# Autodesk Inventor assembly: 1301.000(1)
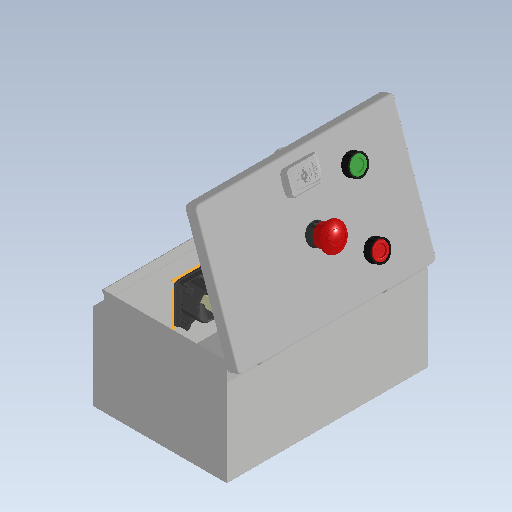
[picture p0: Inventor's stored thumbnail of the model, 512x512]
Saved by Autodesk Inventor 2025.2 (Build 292293000, 293)
## iProperties
Category: PARTsolutions
Company: RITTAL
Created: 2025-05-02
Part Number: 1301.000(1)
Catalog Web Link: www.cadenas.de
Description: KX E-Box-stainless steel
Vendor: RITTAL
Document SubType Name: Assembly
Designer: psAdmin
Manufacturer: RITTAL
Mass: 539.801 g
Surface Area: 7071.18 cm^2
Volume: 539.801 cm^3
PSOL_IDENT_0: {$CADENAS_DATA/23d-libs/rittal/schaltschranksys/edelstahl/kleingehause/eb_edel_2_0_asmtab.prj},188 {
PSOL_IDENT_1: VTYP=3D},{STYP=ASSTAB},{NB=1301.000(1)},{LINA=1301.000},{NN=KX E-Box},{DATE=28.04.2025 21:10:46},{GE
PSOL_IDENT_2: OMDATE=11.04.2025 11:21:28},{VERSION=},{LINEID=690},{WBVAR=DETAIL},{WBNUMERIC=DETAIL}  {NB=1301.000(
PSOL_IDENT_3: 1)},{LINA=1301.000},{KT=DUMMY},{BEST=1301.000},{INFOPAGE=-},{DETAIL=1},{INFOWWW=Website},{BEZ1=KX El
PSOL_IDENT_4: ektronik-Box},{BEZ2=Edelstahl, 1.4404},{BEZ3=eintürig},{B=200},{H=300},{T=155},{F=175},{G=285},{GEW=
PSOL_IDENT_5: 3,889},{INFOPATH=http://www.rittal.com/com-en/part/1301000},{CNSECLASS51=27-18-01-02},{CNSECLASS70=2
PSOL_IDENT_6: 7-18-01-01},{CNSECLASS80=27-18-01-01},{CNSETIM40=EC002713},{PPATH=assemblies_eb_edel_2_0/kx_eb_edel_
PSOL_IDENT_7: new_asmtpl.prj},{BESTE1=1301},{BESTE2=000},{CNSETIM80=EC000261},{CNSETIM90=EC000261},{CNSECLASS60=27
PSOL_IDENT_8: -18-01-01},{UNSPSC=31-26-15-02}
NB: 1301.000(1)
NN: KX E-Box
NT: stainless steel
NBSYN: $BEST.($DETAIL.)
LINA: 1301.000
CATALOG: Rittal
BEST: 1301.000
DETAIL: high
INFOWWW: Website
BEZ1: KX E-Box
BEZ2: Stainless steel, 1.4404
BEZ3: single door
B: 200
H: 300
T: 155
F: 175
G: 285
CNSECLASS70: 27-18-01-01
CNSECLASS80: 27-18-01-01
CNSETIM80: EC000261
CNSETIM90: EC000261
CNSECLASS60: 27-18-01-01
UNSPSC: 31-26-15-02
SUPPLIER: RITTAL
ARTICLENO: 1301.000(1)
BOMINFO: 1301.000
CREATOR: CADENAS GmbH
Title: 1301.000
Author: Cadenas PARTsolutions
Comments: stainless steel
## Documents named in this file (22)
- C:\Users\Gustavo Sousa\Downloads\Inventor\design\quadro_eletrico\AIS2024\1301_000_1_\1301_000(1).iam
- C:\Users\Gustavo Sousa\Downloads\Inventor\design\quadro_eletrico\AIS2024\1301_000_1_\1301_000_1_(1).ipt
- C:\Users\Gustavo Sousa\Downloads\Inventor\design\quadro_eletrico\AIS2024\1301_000_1_\1301_000_6_(1).ipt
- C:\Users\Gustavo Sousa\Downloads\Inventor\design\quadro_eletrico\AIS2024\1301_000_1_\1301_000_4_(1).ipt
- C:\Users\Gustavo Sousa\Downloads\Inventor\design\quadro_eletrico\AIS2024\1301_000_1_\1301_000_2_(1).ipt
- C:\Users\Gustavo Sousa\Downloads\Inventor\design\quadro_eletrico\AIS2024\1301_000_1_\1301_000_5_(1).ipt
- C:\Users\Gustavo Sousa\Downloads\Inventor\design\quadro_eletrico\AIS2024\1301_000_1_\1301_000_3_(1).ipt
- C:\Users\Gustavo Sousa\Downloads\Inventor\design\quadro_eletrico\AIS2024\1301_000_1_\1301_000_10_(1).ipt
- C:\Users\Gustavo Sousa\Downloads\Inventor\design\calhadine\PP0735H(1).ipt
- C:\Users\Gustavo Sousa\Downloads\Inventor\design\disjuntores\Diferencial\CFC 225P\CFC 225P v16\CFC 225P v16\CFC 225P v16.ipt
- C:\Users\Gustavo Sousa\Downloads\Inventor\design\disjuntores\Polares\SD C25 1P - STECK\SD C25 1P - STECK\SD C25 1P - STECK.ipt
- C:\Users\Gustavo Sousa\Downloads\Inventor\design\barramento\MONTAGEM BARRAMENTO 10 FUROS NEUTRO\MONTAGEM BARRAMENTO 10 FUROS NEUTRO\MONTAGEM BARRAMENTO 10 FUROS NEUTRO.ipt
- C:\Users\Gustavo Sousa\Downloads\Inventor\design\barramento\BARRAMENTO 10 FUROS NEUTRO\BARRAMENTO 10 FUROS NEUTRO\BARRAMENTO 10 FUROS NEUTRO.ipt
- C:\Users\Gustavo Sousa\Downloads\Inventor\design\disjuntores\Motor\3RV24111AA200DA0.ipt
- C:\Users\Gustavo Sousa\Downloads\Inventor\design\corte_Geral\AIS2024\5SP33253.iam
- C:\Users\Gustavo Sousa\Downloads\Inventor\design\bornes\280-607_HI_0001_002.ipt
- C:\Users\Gustavo Sousa\Downloads\Inventor\design\bornes\280-607_HI.ipt
- C:\Users\Gustavo Sousa\Downloads\Inventor\design\bornes\280-607_HI_0003_001.ipt
- C:\Users\Gustavo Sousa\Downloads\Inventor\design\botões\P20BKR1\P20BKR1\P20BKR1.ipt
- C:\Users\Gustavo Sousa\Downloads\Inventor\design\botões\botao-lk2-ea42-verde-1nf-cod-14010-1.snapshot.1\MONTAGEM DO BOTÃO3.iam
- C:\Users\Gustavo Sousa\Downloads\Inventor\design\botões\botao-lk2-ea42-vermelho-1.snapshot.1\MONTAGEM DO BOTÃO.iam
- C:\Users\Gustavo Sousa\Downloads\Inventor\design\corte_Geral\eaton-main-switch-p1-25-m4-svb-switch-1.snapshot.1\Eaton main switch P1-25-M4-SVB - switch\Eaton main switch P1-25-M4-SVB - switch\Eaton main switch .ipt
## Components (31 placed, 26 different names)
1. 1301_000_1_(1):1 — to_MP_XY@1 <-> MONTAGEPLATTE_XY@2, to_MP_Z@1 <-> MONTAGEPLATTE_Z@2, to_MP_YZ@1 <-> MONTAGEPLATTE_YZ@2, to_HINGE_1_XY@1 <-> HINGE_XY@3, to_HINGE_1_Z@1 <-> HINGE_Z@3, to_HINGE_1_YZ@1 <-> HINGE_YZ@3, to_HINGE_2_XY@1 <-> HINGE_XY@4, to_HINGE_2_Z@1 <-> HINGE_Z@4, to_HINGE_2_YZ@1 <-> HINGE_YZ@4, to_L_Winkel_Bottom_XY@1 <-> SEITENTEIL_XY@7, to_L_Winkel_Bottom_Z@1 <-> SEITENTEIL_Z@7, to_L_Winkel_Bottom_YZ@1 <-> SEITENTEIL_YZ@7, to_L_Winkel_Top_XY@1 <-> SEITENTEIL_XY@10, to_L_Winkel_Top_Z@1 <-> SEITENTEIL_Z@10, to_L_Winkel_Top_YZ@1 <-> SEITENTEIL_YZ@10, Coincidente:67, Coincidente:68, Coincidente:69
2. 1301_000_6_(1):1 — to_MP_XY@1 <-> MONTAGEPLATTE_XY@2, to_MP_Z@1 <-> MONTAGEPLATTE_Z@2, to_MP_YZ@1 <-> MONTAGEPLATTE_YZ@2, Coincidente:23, Coincidente:24, Coincidente:25, Coincidente:26, Coincidente:27, Coincidente:28
3. 1301_000_4_(1):1 — to_HINGE_1_XY@1 <-> HINGE_XY@3, to_HINGE_1_Z@1 <-> HINGE_Z@3, to_HINGE_1_YZ@1 <-> HINGE_YZ@3
4. 1301_000_4_(1):2 — to_HINGE_2_XY@1 <-> HINGE_XY@4, to_HINGE_2_Z@1 <-> HINGE_Z@4, to_HINGE_2_YZ@1 <-> HINGE_YZ@4, DECKEL_XY@4 <-> to_HINGE_1_XY@5, DECKEL_Z@4 <-> to_HINGE_1_Z@5
5. 1301_000_2_(1):1 — DECKEL_XY@4 <-> to_HINGE_1_XY@5, DECKEL_Z@4 <-> to_HINGE_1_Z@5, VB_XY@5 <-> VV_XY@6, VB_Z@5 <-> VV_Z@6, VB_YZ@5 <-> VV_YZ@6, Coincidente:61, Coincidente:62, Coincidente:63, Coincidente:64, Coincidente:65, Coincidente:66
6. 1301_000_5_(1):1 — VB_XY@5 <-> VV_XY@6, VB_Z@5 <-> VV_Z@6, VB_YZ@5 <-> VV_YZ@6
7. 1301_000_3_(1):1 — to_L_Winkel_Bottom_XY@1 <-> SEITENTEIL_XY@7, to_L_Winkel_Bottom_Z@1 <-> SEITENTEIL_Z@7, to_L_Winkel_Bottom_YZ@1 <-> SEITENTEIL_YZ@7, SC1_XY@7 <-> SCHRAUBE_XY@8, SC1_Z@7 <-> SCHRAUBE_Z@8, SC1_YZ@7 <-> SCHRAUBE_YZ@8, SC2_XY@7 <-> SCHRAUBE_XY@9, SC2_Z@7 <-> SCHRAUBE_Z@9, SC2_YZ@7 <-> SCHRAUBE_YZ@9
8. 1301_000_10_(1):1 — SC1_XY@7 <-> SCHRAUBE_XY@8, SC1_Z@7 <-> SCHRAUBE_Z@8, SC1_YZ@7 <-> SCHRAUBE_YZ@8
9. 1301_000_10_(1):2 — SC2_XY@7 <-> SCHRAUBE_XY@9, SC2_Z@7 <-> SCHRAUBE_Z@9, SC2_YZ@7 <-> SCHRAUBE_YZ@9
10. 1301_000_3_(1):2 — to_L_Winkel_Top_XY@1 <-> SEITENTEIL_XY@10, to_L_Winkel_Top_Z@1 <-> SEITENTEIL_Z@10, to_L_Winkel_Top_YZ@1 <-> SEITENTEIL_YZ@10, SC1_XY@10 <-> SCHRAUBE_XY@11, SC1_Z@10 <-> SCHRAUBE_Z@11, SC1_YZ@10 <-> SCHRAUBE_YZ@11, SC2_XY@10 <-> SCHRAUBE_XY@12, SC2_Z@10 <-> SCHRAUBE_Z@12, SC2_YZ@10 <-> SCHRAUBE_YZ@12
11. 1301_000_10_(1):3 — SC1_XY@10 <-> SCHRAUBE_XY@11, SC1_Z@10 <-> SCHRAUBE_Z@11, SC1_YZ@10 <-> SCHRAUBE_YZ@11
12. 1301_000_10_(1):4 — SC2_XY@10 <-> SCHRAUBE_XY@12, SC2_Z@10 <-> SCHRAUBE_Z@12, SC2_YZ@10 <-> SCHRAUBE_YZ@12
13. calhadine 1 — Coincidente:23, Coincidente:24, Coincidente:25, Coincidente:29, Coincidente:30, Coincidente:31, Coincidente:32, Coincidente:33, Coincidente:34, Coincidente:35, Coincidente:36, Coincidente:37, Coincidente:38, Coincidente:39, Coincidente:40, Coincidente:41, Coincidente:42
14. calhadine 2 — Coincidente:26, Coincidente:27, Coincidente:28, Coincidente:44, Coincidente:45, Coincidente:46, Coincidente:47, Coincidente:49, Coincidente:50, Coincidente:52, Coincidente:53, Coincidente:55, Coincidente:56, Coincidente:57, Coincidente:58, Coincidente:59
15. disjuntor_diferencial — Coincidente:29, Coincidente:30
16. disjuntor_monopolar — Coincidente:31, Coincidente:32
17. barramento_Fase — Coincidente:33, Coincidente:34
18. barramento_Neutro — Coincidente:35, Coincidente:36
19. disjuntor_Motor1 — Coincidente:37, Coincidente:38
20. corte_Geral [sub-assembly] — Coincidente:39, Coincidente:40
21. disjuntor_Motor2 — Coincidente:41, Coincidente:42
22. borne_Viking_Neutro_1.0 — Coincidente:46, Coincidente:47, Coincidente:54
23. borne_Viking_Neutro_2.0 — Coincidente:52, Coincidente:53, Coincidente:54
24. borne_Viking_Fase_2 — Coincidente:44, Coincidente:45, Coincidente:51
25. borne_Viking_Fase_2.1 — Coincidente:49, Coincidente:50, Coincidente:51
26. borne_Viking_Terra_1.0 — Coincidente:55, Coincidente:56, Coincidente:57, Coincidente:60
27. borne_Viking_terra_1.1 — Coincidente:58, Coincidente:59, Coincidente:60
28. botao_emergencia — Coincidente:61, Coincidente:62
29. MONTAGEM DO BOTÃO3:1 [sub-assembly] — Coincidente:63, Coincidente:64
30. MONTAGEM DO BOTÃO:1 [sub-assembly] — Coincidente:65, Coincidente:66
31. Eaton main switch :1 — Coincidente:67, Coincidente:68, Coincidente:69
## Relationships (77: Mate 67, Angle 10)
- to_MP_XY@1 <-> MONTAGEPLATTE_XY@2 [Mate]: 1301_000_1_(1):1 ↔ 1301_000_6_(1):1
- to_MP_Z@1 <-> MONTAGEPLATTE_Z@2 [Mate]: 1301_000_1_(1):1 ↔ 1301_000_6_(1):1
- to_MP_YZ@1 <-> MONTAGEPLATTE_YZ@2 [Angle] (0 deg): 1301_000_1_(1):1 ↔ 1301_000_6_(1):1
- to_HINGE_1_XY@1 <-> HINGE_XY@3 [Mate]: 1301_000_1_(1):1 ↔ 1301_000_4_(1):1
- to_HINGE_1_Z@1 <-> HINGE_Z@3 [Mate]: 1301_000_1_(1):1 ↔ 1301_000_4_(1):1
- to_HINGE_1_YZ@1 <-> HINGE_YZ@3 [Angle] (90 deg): 1301_000_1_(1):1 ↔ 1301_000_4_(1):1
- to_HINGE_2_XY@1 <-> HINGE_XY@4 [Mate]: 1301_000_1_(1):1 ↔ 1301_000_4_(1):2
- to_HINGE_2_Z@1 <-> HINGE_Z@4 [Mate]: 1301_000_1_(1):1 ↔ 1301_000_4_(1):2
- to_HINGE_2_YZ@1 <-> HINGE_YZ@4 [Angle] (90 deg): 1301_000_1_(1):1 ↔ 1301_000_4_(1):2
- DECKEL_XY@4 <-> to_HINGE_1_XY@5 [Mate]: 1301_000_4_(1):2 ↔ 1301_000_2_(1):1
- DECKEL_Z@4 <-> to_HINGE_1_Z@5 [Mate]: 1301_000_4_(1):2 ↔ 1301_000_2_(1):1
- VB_XY@5 <-> VV_XY@6 [Mate]: 1301_000_2_(1):1 ↔ 1301_000_5_(1):1
- VB_Z@5 <-> VV_Z@6 [Mate]: 1301_000_2_(1):1 ↔ 1301_000_5_(1):1
- VB_YZ@5 <-> VV_YZ@6 [Angle] (0 deg): 1301_000_2_(1):1 ↔ 1301_000_5_(1):1
- to_L_Winkel_Bottom_XY@1 <-> SEITENTEIL_XY@7 [Mate] (-0.25 mm): 1301_000_1_(1):1 ↔ 1301_000_3_(1):1
- to_L_Winkel_Bottom_Z@1 <-> SEITENTEIL_Z@7 [Mate]: 1301_000_1_(1):1 ↔ 1301_000_3_(1):1
- to_L_Winkel_Bottom_YZ@1 <-> SEITENTEIL_YZ@7 [Angle] (-90 deg): 1301_000_1_(1):1 ↔ 1301_000_3_(1):1
- SC1_XY@7 <-> SCHRAUBE_XY@8 [Mate] (-1.575 mm): 1301_000_3_(1):1 ↔ 1301_000_10_(1):1
- SC1_Z@7 <-> SCHRAUBE_Z@8 [Mate]: 1301_000_3_(1):1 ↔ 1301_000_10_(1):1
- SC1_YZ@7 <-> SCHRAUBE_YZ@8 [Angle] (0 deg): 1301_000_3_(1):1 ↔ 1301_000_10_(1):1
- SC2_XY@7 <-> SCHRAUBE_XY@9 [Mate] (-1.575 mm): 1301_000_3_(1):1 ↔ 1301_000_10_(1):2
- SC2_Z@7 <-> SCHRAUBE_Z@9 [Mate]: 1301_000_3_(1):1 ↔ 1301_000_10_(1):2
- SC2_YZ@7 <-> SCHRAUBE_YZ@9 [Angle] (0 deg): 1301_000_3_(1):1 ↔ 1301_000_10_(1):2
- to_L_Winkel_Top_XY@1 <-> SEITENTEIL_XY@10 [Mate] (-0.25 mm): 1301_000_1_(1):1 ↔ 1301_000_3_(1):2
- to_L_Winkel_Top_Z@1 <-> SEITENTEIL_Z@10 [Mate]: 1301_000_1_(1):1 ↔ 1301_000_3_(1):2
- to_L_Winkel_Top_YZ@1 <-> SEITENTEIL_YZ@10 [Angle] (90 deg): 1301_000_1_(1):1 ↔ 1301_000_3_(1):2
- SC1_XY@10 <-> SCHRAUBE_XY@11 [Mate] (-1.575 mm): 1301_000_3_(1):2 ↔ 1301_000_10_(1):3
- SC1_Z@10 <-> SCHRAUBE_Z@11 [Mate]: 1301_000_3_(1):2 ↔ 1301_000_10_(1):3
- SC1_YZ@10 <-> SCHRAUBE_YZ@11 [Angle] (0 deg): 1301_000_3_(1):2 ↔ 1301_000_10_(1):3
- SC2_XY@10 <-> SCHRAUBE_XY@12 [Mate] (-1.575 mm): 1301_000_3_(1):2 ↔ 1301_000_10_(1):4
- SC2_Z@10 <-> SCHRAUBE_Z@12 [Mate]: 1301_000_3_(1):2 ↔ 1301_000_10_(1):4
- SC2_YZ@10 <-> SCHRAUBE_YZ@12 [Angle] (0 deg): 1301_000_3_(1):2 ↔ 1301_000_10_(1):4
- Coincidente:23 [Mate]: 1301_000_6_(1):1 ↔ calhadine 1
- Coincidente:24 [Mate]: 1301_000_6_(1):1 ↔ calhadine 1
- Coincidente:25 [Mate] (0.128 mm): 1301_000_6_(1):1 ↔ calhadine 1
- Coincidente:26 [Mate]: 1301_000_6_(1):1 ↔ calhadine 2
- Coincidente:27 [Mate]: 1301_000_6_(1):1 ↔ calhadine 2
- Coincidente:28 [Mate] (0.156 mm): 1301_000_6_(1):1 ↔ calhadine 2
- Coincidente:29 [Mate]: calhadine 1 ↔ disjuntor_diferencial
- Coincidente:30 [Mate]: calhadine 1 ↔ disjuntor_diferencial
- Coincidente:31 [Mate]: calhadine 1 ↔ disjuntor_monopolar
- Coincidente:32 [Mate]: calhadine 1 ↔ disjuntor_monopolar
- Coincidente:33 [Mate]: calhadine 1 ↔ barramento_Fase
- Coincidente:34 [Mate]: calhadine 1 ↔ barramento_Fase
- Coincidente:35 [Mate]: calhadine 1 ↔ barramento_Neutro
- Coincidente:36 [Mate]: calhadine 1 ↔ barramento_Neutro
- Coincidente:37 [Mate]: calhadine 1 ↔ disjuntor_Motor1
- Coincidente:38 [Mate]: calhadine 1 ↔ disjuntor_Motor1
- Coincidente:39 [Mate]: calhadine 1 ↔ corte_Geral
- Coincidente:40 [Mate]: calhadine 1 ↔ corte_Geral
- Coincidente:41 [Mate]: calhadine 1 ↔ disjuntor_Motor2
- Coincidente:42 [Mate]: calhadine 1 ↔ disjuntor_Motor2
- Coincidente:44 [Mate]: calhadine 2 ↔ borne_Viking_Fase_2
- Coincidente:45 [Mate]: calhadine 2 ↔ borne_Viking_Fase_2
- Coincidente:46 [Mate]: calhadine 2 ↔ borne_Viking_Neutro_1.0
- Coincidente:47 [Mate]: calhadine 2 ↔ borne_Viking_Neutro_1.0
- Coincidente:49 [Mate]: calhadine 2 ↔ borne_Viking_Fase_2.1
- Coincidente:50 [Mate]: calhadine 2 ↔ borne_Viking_Fase_2.1
- Coincidente:51 [Mate]: borne_Viking_Fase_2 ↔ borne_Viking_Fase_2.1
- Coincidente:52 [Mate]: calhadine 2 ↔ borne_Viking_Neutro_2.0
- Coincidente:53 [Mate]: calhadine 2 ↔ borne_Viking_Neutro_2.0
- Coincidente:54 [Mate]: borne_Viking_Neutro_1.0 ↔ borne_Viking_Neutro_2.0
- Coincidente:55 [Mate]: calhadine 2 ↔ borne_Viking_Terra_1.0
- Coincidente:56 [Mate]: calhadine 2 ↔ borne_Viking_Terra_1.0
- Coincidente:57 [Mate]: calhadine 2 ↔ borne_Viking_Terra_1.0
- Coincidente:58 [Mate]: calhadine 2 ↔ borne_Viking_terra_1.1
- Coincidente:59 [Mate]: calhadine 2 ↔ borne_Viking_terra_1.1
- Coincidente:60 [Mate]: borne_Viking_Terra_1.0 ↔ borne_Viking_terra_1.1
- Coincidente:61 [Mate]: 1301_000_2_(1):1 ↔ botao_emergencia
- Coincidente:62 [Mate]: 1301_000_2_(1):1 ↔ botao_emergencia
- Coincidente:63 [Mate]: 1301_000_2_(1):1 ↔ MONTAGEM DO BOTÃO3:1
- Coincidente:64 [Mate]: 1301_000_2_(1):1 ↔ MONTAGEM DO BOTÃO3:1
- Coincidente:65 [Mate]: 1301_000_2_(1):1 ↔ MONTAGEM DO BOTÃO:1
- Coincidente:66 [Mate]: 1301_000_2_(1):1 ↔ MONTAGEM DO BOTÃO:1
- Coincidente:67 [Mate]: 1301_000_1_(1):1 ↔ Eaton main switch :1
- Coincidente:68 [Mate]: 1301_000_1_(1):1 ↔ Eaton main switch :1
- Coincidente:69 [Mate]: 1301_000_1_(1):1 ↔ Eaton main switch :1
